# Autodesk Inventor assembly: Gotowa przekładnia
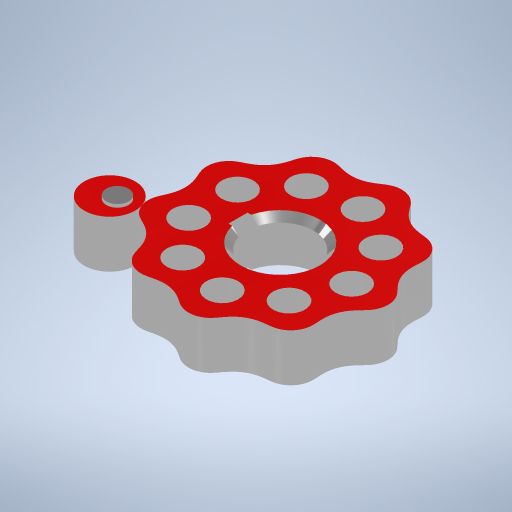
[picture p0: Inventor's stored thumbnail of the model, 512x512]
Saved by Autodesk Inventor 2023 (Build 270158000, 158)
## iProperties
Created: 2023-04-01
Part Number: Gotowa przekładnia
Document SubType Name: Assembly
Designer: Wiktor
Author: Wiktor
## Documents named in this file (3)
- C:\Users\Wiktor\Documents\Manipulator\Gotowa przekładnia.iam
- C:\Users\Wiktor\Documents\Manipulator\Przekładnia cykloidalna mimośrodowa.ipt
- C:\Users\Wiktor\Documents\Manipulator\Przekładnia rolka.ipt
## Components (2 placed, 2 different names)
1. Przekładnia cykloidalna mimośrodowa:1 — Równoległe:1, Zestawiające:1, Zestawiające:2
2. Przekładnia rolka:1 — Równoległe:1, Zestawiające:1, Zestawiające:2
## Relationships (3: Mate 2, Flush 1)
- Równoległe:1 [Flush]: Przekładnia cykloidalna mimośrodowa:1 ↔ Przekładnia rolka:1
- Zestawiające:1 [Mate] (40 mm): Przekładnia cykloidalna mimośrodowa:1 ↔ Przekładnia rolka:1
- Zestawiające:2 [Mate] (40 mm): Przekładnia cykloidalna mimośrodowa:1 ↔ Przekładnia rolka:1
